# Autodesk Inventor assembly: Screw Jack Asembly
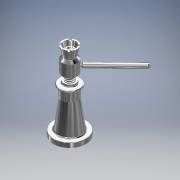
[picture p0: Inventor's stored thumbnail of the model, 180x180]
Saved by Autodesk Inventor 2018 (Build 220112000, 112)
## iProperties
Created: 2019-08-31
Part Number: Screw Jack Asembly
Document SubType Name: Assembly
Designer: HP
Author: HP
## Documents named in this file (8)
- C:\Users\Sameer\Desktop\Saad\SMA\Screw Jack\Screw Jack Asembly.iam
- C:\Users\Sameer\Desktop\Saad\SMA\Screw Jack\Screw jack.ipt
- C:\Users\Sameer\Desktop\Saad\SMA\Screw Jack\Nut of Screw Jack.ipt
- C:\Users\Sameer\Desktop\Saad\SMA\Screw Jack\Spindle.ipt
- C:\Users\Sameer\Desktop\Saad\SMA\Screw Jack\Screw Jack Cup.ipt
- C:\Users\Sameer\Desktop\Saad\SMA\Screw Jack\Washer.ipt
- C:\Users\Sameer\Desktop\Saad\SMA\Screw Jack\Screw.ipt
- C:\Users\Sameer\Desktop\Saad\SMA\Screw Jack\Tommy Bar.ipt
## Components (7 placed, 7 different names)
1. Screw jack:1 — Mate:1, Mate:2
2. Nut of Screw Jack:1 — Mate:1, Mate:2, Mate:3, Mate:4
3. Spindle:1 — Mate:3, Mate:4, Mate:5, Mate:8, Mate:9
4. Screw Jack Cup:1 — Mate:5
5. Washer:1
6. Screw:1 — Mate:8
7. Tommy Bar:1 — Mate:9
## Relationships (7: Mate 7)
- Mate:1: Screw jack:1 ↔ Nut of Screw Jack:1
- Mate:2: Screw jack:1 ↔ Nut of Screw Jack:1
- Mate:3: Nut of Screw Jack:1 ↔ Spindle:1
- Mate:4 (20 mm): Nut of Screw Jack:1 ↔ Spindle:1
- Mate:5: Spindle:1 ↔ Screw Jack Cup:1
- Mate:8: Spindle:1 ↔ Screw:1
- Mate:9: Spindle:1 ↔ Tommy Bar:1
